# Autodesk Inventor assembly: poleStandHorizAssyB
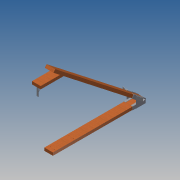
[picture p0: Inventor's stored thumbnail of the model, 180x180]
Saved by Autodesk Inventor 2014 SP1 (Build 180222100, 222)
## iProperties
Created: 2014-08-25
Part Number: poleStandHorizAssyB
Document SubType Name: Assembly
Designer: Dave
Author: Dave
## Documents named in this file (7)
- C:\Users\Dave\Desktop\hera-cad\support\pole\poleStandHorizAssy.iam
- C:\Users\Dave\Desktop\hera-cad\support\pole\poleStandHoriz2.ipt
- C:\Users\Dave\Desktop\hera-cad\support\pole\poleStand37.ipt
- C:\Users\Dave\Desktop\hera-cad\support\pole\poleStandHoriz3.ipt
- C:\Users\Dave\Desktop\hera-cad\smallParts\angleBracket.ipt
- C:\Users\Dave\Desktop\hera-cad\support\endcaps\HERA_end_cap_left.iam
- C:\Users\Dave\Desktop\hera-cad\support\endcaps\HERA_end_cap_right.iam
## Components (6 placed, 6 different names)
1. HERA_end_cap_left:1 [sub-assembly] — Mate:9, Mate:10, Flush:3, Mate:11, Mate:12, Flush:4
2. poleStandHoriz2:1 — Mate:9, Mate:10, Flush:3, Flush:6
3. poleStand37:1 — Mate:7, Flush:1, Mate:11, Mate:12, Flush:4, Mate:13, Mate:14, Flush:5
4. poleStandHoriz3:1 — Mate:7, Flush:1, Mate:8, Flush:2, Flush:6
5. angleBracket:1 — Mate:8, Flush:2
6. HERA_end_cap_right:1 [sub-assembly] — Mate:13, Mate:14, Flush:5
## Relationships (14: Mate 8, Flush 6)
- Mate:7: poleStand37:1 ↔ poleStandHoriz3:1
- Flush:1: poleStand37:1 ↔ poleStandHoriz3:1
- Mate:8: poleStandHoriz3:1 ↔ angleBracket:1
- Flush:2: poleStandHoriz3:1 ↔ angleBracket:1
- Mate:9: HERA_end_cap_left:1 ↔ poleStandHoriz2:1
- Mate:10: HERA_end_cap_left:1 ↔ poleStandHoriz2:1
- Flush:3 (37 mm): HERA_end_cap_left:1 ↔ poleStandHoriz2:1
- Mate:11: HERA_end_cap_left:1 ↔ poleStand37:1
- Mate:12: HERA_end_cap_left:1 ↔ poleStand37:1
- Flush:4: HERA_end_cap_left:1 ↔ poleStand37:1
- Mate:13: poleStand37:1 ↔ HERA_end_cap_right:1
- Mate:14: poleStand37:1 ↔ HERA_end_cap_right:1
- Flush:5: poleStand37:1 ↔ HERA_end_cap_right:1
- Flush:6 (-162.56 mm): poleStandHoriz2:1 ↔ poleStandHoriz3:1
